# Autodesk Inventor assembly: Assembly1
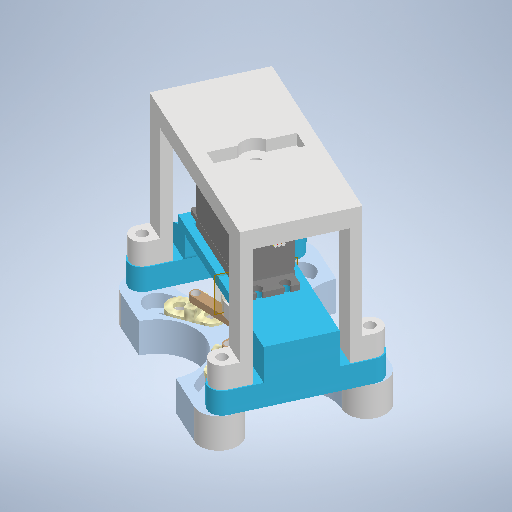
[picture p0: Inventor's stored thumbnail of the model, 512x512]
Saved by Autodesk Inventor 2025.1 (Build 291241000, 241)
## iProperties
Created: 2024-10-07
Part Number: Assembly1
Document SubType Name: Assembly
Designer: m_kni
Author: m_kni
## Documents named in this file (9)
- C:\Users\m_kni\OneDrive\Documents\GitHub\Perovskite-Automated-Synthesis-System\CAD\Gripper\Assembly1.iam
- C:\Users\m_kni\OneDrive\Documents\GitHub\Perovskite-Automated-Synthesis-System\CAD\Gripper\BaseSketchGrabberrev2.0.ipt
- C:\Users\m_kni\OneDrive\Documents\GitHub\Perovskite-Automated-Synthesis-System\CAD\Gripper\spinner.ipt
- C:\Users\m_kni\OneDrive\Documents\GitHub\Perovskite-Automated-Synthesis-System\CAD\Gripper\5x5x11bearing.ipt
- C:\Users\m_kni\OneDrive\Documents\GitHub\Perovskite-Automated-Synthesis-System\CAD\Gripper\bearing plate.ipt
- C:\Users\m_kni\OneDrive\Documents\GitHub\Perovskite-Automated-Synthesis-System\CAD\Gripper\link.ipt
- C:\Users\m_kni\OneDrive\Documents\GitHub\Perovskite-Automated-Synthesis-System\CAD\Non 3D Printed Parts\Motors and Servos\Servo MG996R.ipt
- C:\Users\m_kni\OneDrive\Documents\GitHub\Perovskite-Automated-Synthesis-System\CAD\Gripper\SERVO_MOUNT_TOBASE.ipt
- C:\Users\m_kni\OneDrive\Documents\GitHub\Perovskite-Automated-Synthesis-System\CAD\Gripper\ATTACHMENT_TOOLHEAD_GRIPPER.ipt
## Components (22 placed, 8 different names)
1. BaseSketchGrabberrev2.0:1 — Insert:1, Insert:5, Tangent:1, Insert:7, Mate:1, Insert:10, Mate:2, Insert:13, Mate:3, Angle:1, Insert:17, Insert:18
2. spinner:1 — Insert:2, Rotational:1, Rotational:2, Rotational:5, Rotational:7, Insert:16
3. 5x5x11bearing:1 — Insert:1, Insert:2
4. bearing plate:1 — Insert:3, Insert:4, Insert:6
5. 5x5x11bearing:2 — Insert:3, Tangent:1
6. 5x5x11bearing:3 — Insert:4, Insert:5
7. link:1 — Insert:6, Rotational:1
8. 5x5x11bearing:4 — Insert:7, Insert:8
9. 5x5x11bearing:5 — Insert:9
10. bearing plate:2 — Insert:8, Mate:1, Insert:9, Rotational:3
11. link:2 — Rotational:2, Rotational:3
12. 5x5x11bearing:6 — Insert:10, Insert:11
13. bearing plate:3 — Insert:11, Mate:2, Insert:12, Rotational:4
14. 5x5x11bearing:7 — Insert:12
15. 5x5x11bearing:8 — Insert:13, Insert:14
16. bearing plate:4 — Insert:14, Mate:3, Insert:15, Rotational:6
17. 5x5x11bearing:9 — Insert:15
18. link:3 — Rotational:4, Rotational:5
19. link:4 — Rotational:6, Rotational:7
20. Servo MG996R:1 — Insert:16, Angle:1
21. SERVO_MOUNT_TOBASE:1 — Insert:17, Insert:18, Insert:19, Insert:20
22. ATTACHMENT_TOOLHEAD_GRIPPER:1 — Insert:19, Insert:20
## Relationships (32: Insert 20, RevoluteJoint 7, Mate 3, Tangent 1, Angle 1)
- Insert:1: BaseSketchGrabberrev2.0:1 ↔ 5x5x11bearing:1
- Insert:2: spinner:1 ↔ 5x5x11bearing:1
- Insert:3: bearing plate:1 ↔ 5x5x11bearing:2
- Insert:4: bearing plate:1 ↔ 5x5x11bearing:3
- Insert:5: BaseSketchGrabberrev2.0:1 ↔ 5x5x11bearing:3
- Tangent:1: BaseSketchGrabberrev2.0:1 ↔ 5x5x11bearing:2
- Insert:6: bearing plate:1 ↔ link:1
- Rotational:1 [RevoluteJoint]: spinner:1 ↔ link:1
- Insert:7: BaseSketchGrabberrev2.0:1 ↔ 5x5x11bearing:4
- Insert:8: 5x5x11bearing:4 ↔ bearing plate:2
- Mate:1: BaseSketchGrabberrev2.0:1 ↔ bearing plate:2
- Insert:9: 5x5x11bearing:5 ↔ bearing plate:2
- Rotational:2 [RevoluteJoint]: spinner:1 ↔ link:2
- Rotational:3 [RevoluteJoint]: bearing plate:2 ↔ link:2
- Insert:10: BaseSketchGrabberrev2.0:1 ↔ 5x5x11bearing:6
- Insert:11: 5x5x11bearing:6 ↔ bearing plate:3
- Mate:2: BaseSketchGrabberrev2.0:1 ↔ bearing plate:3
- Insert:12: bearing plate:3 ↔ 5x5x11bearing:7
- Insert:13: BaseSketchGrabberrev2.0:1 ↔ 5x5x11bearing:8
- Insert:14: 5x5x11bearing:8 ↔ bearing plate:4
- Mate:3: BaseSketchGrabberrev2.0:1 ↔ bearing plate:4
- Insert:15: bearing plate:4 ↔ 5x5x11bearing:9
- Rotational:4 [RevoluteJoint]: bearing plate:3 ↔ link:3
- Rotational:5 [RevoluteJoint]: spinner:1 ↔ link:3
- Rotational:6 [RevoluteJoint]: bearing plate:4 ↔ link:4
- Rotational:7 [RevoluteJoint]: spinner:1 ↔ link:4
- Insert:16 (-2.54 mm): spinner:1 ↔ Servo MG996R:1
- Angle:1 (0 deg): BaseSketchGrabberrev2.0:1 ↔ Servo MG996R:1
- Insert:17: BaseSketchGrabberrev2.0:1 ↔ SERVO_MOUNT_TOBASE:1
- Insert:18: BaseSketchGrabberrev2.0:1 ↔ SERVO_MOUNT_TOBASE:1
- Insert:19: SERVO_MOUNT_TOBASE:1 ↔ ATTACHMENT_TOOLHEAD_GRIPPER:1
- Insert:20: SERVO_MOUNT_TOBASE:1 ↔ ATTACHMENT_TOOLHEAD_GRIPPER:1
